# Autodesk Inventor assembly: CAR_040_NewKickerAssembly
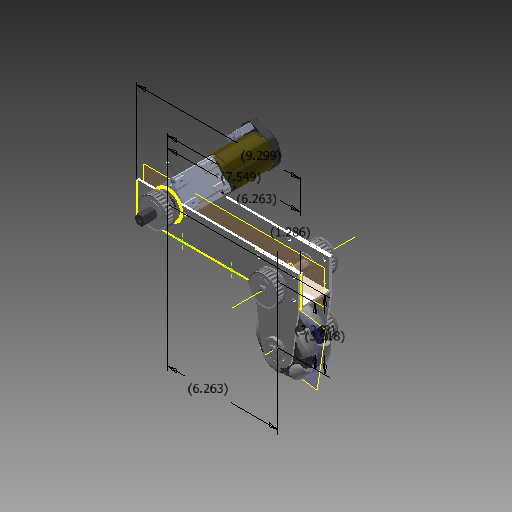
[picture p0: Inventor's stored thumbnail of the model, 512x512]
Saved by Autodesk Inventor 2018.3 (Build 223284000, 284)
## iProperties
Created: 2020-02-13
Part Number: CAR_040_NewKickerAssembly
Document SubType Name: Assembly
Designer: user
Author: user
## Documents named in this file (9)
- C:\Users\myerpaul\Documents\GrabCAD\Infinite Recharge 2020\Build season\CAR_040_NewKickerAssembly.iam
- C:\Users\myerpaul\Documents\GrabCAD\Infinite Recharge 2020\Build season\3 inch OmniWheel STEP\3_25_Omni-Directional_Wheel_217-4775.iam
- C:\Users\myerpaul\Documents\GrabCAD\Infinite Recharge 2020\Build season\CAR_041_KickerGusset.ipt
- C:\Users\myerpaul\Documents\GrabCAD\Infinite Recharge 2020\Build season\DGB STEP\217-4006_0_500_flanged_thunderhex_bearing.ipt
- C:\Users\myerpaul\Documents\GrabCAD\Infinite Recharge 2020\Build season\CAR_042_KickerUChannel.ipt
- C:\Users\myerpaul\Documents\GrabCAD\Infinite Recharge 2020\Brainstorming\Versaplanetary\Versa+Motor.iam
- C:\Users\myerpaul\Documents\GrabCAD\Infinite Recharge 2020\Build season\CAR_043_SDP_a_6a55m024df0910.ipt
- C:\Users\myerpaul\Documents\GrabCAD\Infinite Recharge 2020\Build season\CAR_029_KickerAxle.ipt
- C:\Users\myerpaul\Documents\GrabCAD\Infinite Recharge 2020\Build season\CAR_052_OmniWheelKickerAxle.ipt
## Components (15 placed, 8 different names)
1. CAR_042_KickerUChannel:1 — Insert:1, Mate:17, Mate:24, Mate:25, Flush:4, Mate:31, Mate:32, Flush:5, Mate:36
2. CAR_041_KickerGusset:1 — Mate:2, Mate:24, Mate:32, Flush:5, Insert:3, Insert:4
3. CAR_041_KickerGusset:2 — Mate:25, Flush:4, Mate:31, Insert:2, Insert:5
4. 217-4006_0_500_flanged_thunderhex_bearing:1 — Mate:23, Insert:5, Mate:35, Mate:37, Flush:8
5. 217-4006_0_500_flanged_thunderhex_bearing:2 — Insert:4
6. Versa+Motor:1 [sub-assembly] — Insert:1, Mate:17, Mate:22
7. CAR_043_SDP_a_6a55m024df0910:1 — Mate:22, Mate:36, Flush:10
8. CAR_043_SDP_a_6a55m024df0910:2 — Mate:23, Mate:30, Flush:7, Flush:9
9. CAR_052_OmniWheelKickerAxle:1 — Mate:30, Flush:8, Flush:9
10. 217-4006_0_500_flanged_thunderhex_bearing:3 — Insert:3, Mate:33
11. 217-4006_0_500_flanged_thunderhex_bearing:4 — Insert:2, Mate:38
12. CAR_043_SDP_a_6a55m024df0910:3 — Flush:7, Insert:6, Mate:33
13. CAR_043_SDP_a_6a55m024df0910:4 — Mate:38, Flush:10
14. CAR_029_KickerAxle:2 — Insert:6
15. 3_25_Omni-Directional_Wheel_217-4775:1 [sub-assembly] — Mate:2, Mate:35, Mate:37
## Relationships (26: Mate 14, Insert 6, Flush 6)
- Mate:2: CAR_041_KickerGusset:1 ↔ 3_25_Omni-Directional_Wheel_217-4775:1
- Insert:1: CAR_042_KickerUChannel:1 ↔ Versa+Motor:1
- Mate:17: CAR_042_KickerUChannel:1 ↔ Versa+Motor:1
- Mate:22: Versa+Motor:1 ↔ CAR_043_SDP_a_6a55m024df0910:1
- Mate:23: 217-4006_0_500_flanged_thunderhex_bearing:1 ↔ CAR_043_SDP_a_6a55m024df0910:2
- Mate:24: CAR_042_KickerUChannel:1 ↔ CAR_041_KickerGusset:1
- Mate:25: CAR_042_KickerUChannel:1 ↔ CAR_041_KickerGusset:2
- Mate:30: CAR_043_SDP_a_6a55m024df0910:2 ↔ CAR_052_OmniWheelKickerAxle:1
- Flush:4: CAR_042_KickerUChannel:1 ↔ CAR_041_KickerGusset:2
- Mate:31: CAR_042_KickerUChannel:1 ↔ CAR_041_KickerGusset:2
- Mate:32: CAR_042_KickerUChannel:1 ↔ CAR_041_KickerGusset:1
- Flush:5: CAR_042_KickerUChannel:1 ↔ CAR_041_KickerGusset:1
- Insert:2: CAR_041_KickerGusset:2 ↔ 217-4006_0_500_flanged_thunderhex_bearing:4
- Insert:3: CAR_041_KickerGusset:1 ↔ 217-4006_0_500_flanged_thunderhex_bearing:3
- Insert:4: CAR_041_KickerGusset:1 ↔ 217-4006_0_500_flanged_thunderhex_bearing:2
- Insert:5: CAR_041_KickerGusset:2 ↔ 217-4006_0_500_flanged_thunderhex_bearing:1
- Flush:7: CAR_043_SDP_a_6a55m024df0910:2 ↔ CAR_043_SDP_a_6a55m024df0910:3
- Insert:6: CAR_043_SDP_a_6a55m024df0910:3 ↔ CAR_029_KickerAxle:2
- Mate:33: 217-4006_0_500_flanged_thunderhex_bearing:3 ↔ CAR_043_SDP_a_6a55m024df0910:3
- Mate:35: 217-4006_0_500_flanged_thunderhex_bearing:1 ↔ 3_25_Omni-Directional_Wheel_217-4775:1
- Mate:36 (7.9375 mm): CAR_042_KickerUChannel:1 ↔ CAR_043_SDP_a_6a55m024df0910:1
- Mate:37 (3.175 mm): 217-4006_0_500_flanged_thunderhex_bearing:1 ↔ 3_25_Omni-Directional_Wheel_217-4775:1
- Flush:8: 217-4006_0_500_flanged_thunderhex_bearing:1 ↔ CAR_052_OmniWheelKickerAxle:1
- Flush:9: CAR_043_SDP_a_6a55m024df0910:2 ↔ CAR_052_OmniWheelKickerAxle:1
- Mate:38: 217-4006_0_500_flanged_thunderhex_bearing:4 ↔ CAR_043_SDP_a_6a55m024df0910:4
- Flush:10: CAR_043_SDP_a_6a55m024df0910:1 ↔ CAR_043_SDP_a_6a55m024df0910:4
